# Autodesk Inventor assembly: brake-lever
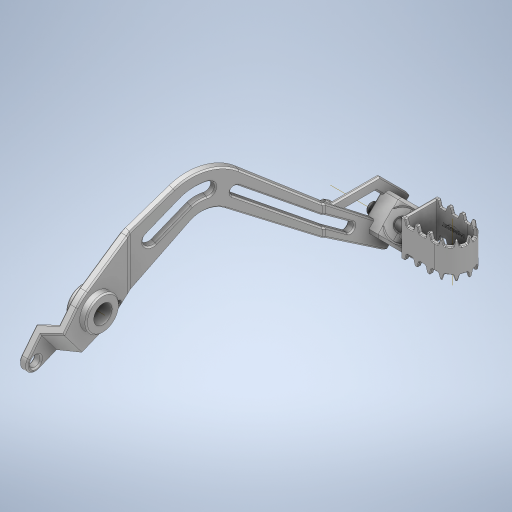
[picture p0: Inventor's stored thumbnail of the model, 512x512]
Saved by Autodesk Inventor 2024 (Build 280153000, 153)
## iProperties
Created: 2023-09-04
Part Number: brake-lever
Document SubType Name: Assembly
Designer: nicx5
Author: nicx5
## Documents named in this file (4)
- E:\Works\Tiger GT 刹车\brake-lever.iam
- E:\Works\Tiger GT 刹车\brake-main.ipt
- E:\Works\Tiger GT 刹车\step-on.ipt
- E:\Works\Tiger GT 刹车\knob.ipt
## Components (3 placed, 3 different names)
1. brake-main:1 — 表面齐平:1, 配合:1, 配合:2, 配合:3, 配合:4, 配合:5, 配合:6
2. step-on:1 — 配合:1, 配合:2, 配合:3, 配合:4, 配合:5, 配合:6, 配合:7
3. knob:1 — 配合:7
## Relationships (8: Mate 7, Flush 1)
- 表面齐平:1 [Flush]: brake-main:1
- 配合:1 [Mate]: brake-main:1 ↔ step-on:1
- 配合:2 [Mate]: brake-main:1 ↔ step-on:1
- 配合:3 [Mate]: brake-main:1 ↔ step-on:1
- 配合:4 [Mate]: brake-main:1 ↔ step-on:1
- 配合:5 [Mate]: brake-main:1 ↔ step-on:1
- 配合:6 [Mate]: brake-main:1 ↔ step-on:1
- 配合:7 [Mate]: step-on:1 ↔ knob:1
